# Autodesk Inventor assembly: MeasurementChamber V4 - SimulationAssembly
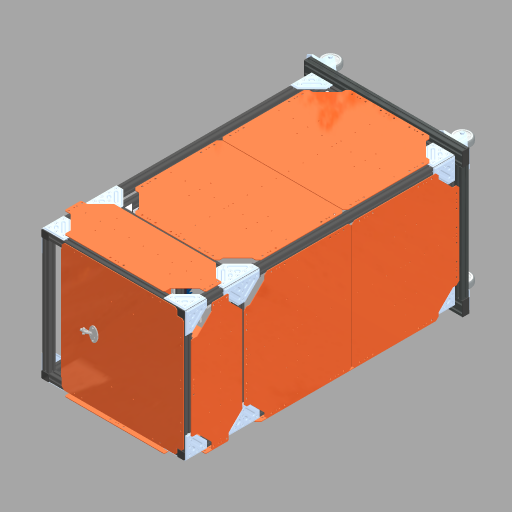
[picture p0: Inventor's stored thumbnail of the model, 512x512]
Saved by Autodesk Inventor 2023 (Build 270158000, 158)
## iProperties
Created: 2024-02-07
Part Number: MeasurementChamber V4 - SimulationAssembly
Document SubType Name: Assembly
Designer: Nils Bade
Mass: 78312.5 g
Surface Area: 384225 cm^2
Volume: 71597.2 cm^3
Density: 1.09379 g/cm^3
Author: Nils Bade
## Documents named in this file (39)
- C:\Users\Nils Bade\Documents\Projektarbeit_Bade\GIT\Masterarbeit-Inventor\RatRig_Bade\Simulation-3D-Models\MeasurementChamber V4 - SimulationAssembly.iam
- C:\Users\Nils Bade\Documents\Projektarbeit_Bade\GIT\Masterarbeit-Inventor\ITEM\ITEM Frame Assembly - Bade v1.iam
- ITEM Frame Assembly - Bade v1.iam
- C:\Users\Nils Bade\Documents\Projektarbeit_Bade\GIT\Masterarbeit-Inventor\RatRig_Bade\Z-Axis Transmission Assembly Back.iam
- C:\Users\Nils Bade\Documents\Projektarbeit_Bade\GIT\Masterarbeit-Inventor\RatRig_Bade\Z-Axis Transmission Assembly Front.iam
- C:\Users\Nils Bade\Documents\Projektarbeit_Bade\GIT\Masterarbeit-Inventor\RatRig_modified\Lead Screw - TR8x8-2p 1057mm Simple.ipt
- C:\Users\Nils Bade\Documents\Projektarbeit_Bade\GIT\Masterarbeit-Inventor\RatRig_modified\Leadscrew Constraint Front for 4040 - Assembly.iam
- C:\Users\Nils Bade\Documents\Projektarbeit_Bade\GIT\Masterarbeit-Inventor\RatRig_modified\Leadscrew Constraint Rear for 4040 - Assembly.iam
- C:\Users\Nils Bade\Documents\Projektarbeit_Bade\GIT\Masterarbeit-Inventor\RatRig_Bade\Bed Arm Back for 4040 - Assembly.iam
- C:\Users\Nils Bade\Documents\Projektarbeit_Bade\GIT\Masterarbeit-Inventor\RatRig_Bade\Bed Arm Left for 4040 - Assembly.iam
- C:\Users\Nils Bade\Documents\Projektarbeit_Bade\GIT\Masterarbeit-Inventor\RatRig_Bade\Bed Arm Right for 4040 - Assembly.iam
- C:\Users\Nils Bade\Documents\Projektarbeit_Bade\GIT\Masterarbeit-Inventor\RatRig_Bade\RatRig-Bade-BedAssembly.iam
- C:\Users\Nils Bade\Documents\Projektarbeit_Bade\GIT\Masterarbeit-Inventor\RatRig_Bade\CoreXY Idler 4040 Assembly Left V2.iam
- C:\Users\Nils Bade\Documents\Projektarbeit_Bade\GIT\Masterarbeit-Inventor\RatRig_Bade\CoreXY Idler 4040 Assembly Right V2.iam
- C:\Users\Nils Bade\Documents\Projektarbeit_Bade\GIT\Masterarbeit-Inventor\RatRig_Bade\CoreXY Motor Assembly Left for 4040 - V3.iam
- C:\Users\Nils Bade\Documents\Projektarbeit_Bade\GIT\Masterarbeit-Inventor\RatRig_Bade\CoreXY Motor Assembly Right for 4040 - V3.iam
- C:\Users\Nils Bade\Documents\Projektarbeit_Bade\GIT\Masterarbeit-Inventor\RatRig_Bade\CoreXY Belts - modified Bade.ipt
- C:\Users\Nils Bade\Documents\Projektarbeit_Bade\GIT\Masterarbeit-Inventor\RatRig_Bade\X-Gantry Assembly for 4040 V3.iam
- C:\Users\Nils Bade\Documents\Projektarbeit_Bade\GIT\Masterarbeit-Inventor\Enclosure\enc - FrontPanel Oben V2 - Assembly.iam
- C:\Users\Nils Bade\Documents\Projektarbeit_Bade\GIT\Masterarbeit-Inventor\Enclosure\enc - SidePanel Oben V2 - Assembly.iam
- C:\Users\Nils Bade\Documents\Projektarbeit_Bade\GIT\Masterarbeit-Inventor\Enclosure\enc-FrontPanel Unten - Assembly no Absorber.iam
- C:\Users\Nils Bade\Documents\Projektarbeit_Bade\GIT\Masterarbeit-Inventor\Enclosure\enc-SidePanel Unten - Assembly no Absorber.iam
- C:\Users\Nils Bade\Documents\Projektarbeit_Bade\GIT\Masterarbeit-Inventor\Enclosure\enc-BackPanel Unten - Assembly.iam
- C:\Users\Nils Bade\Documents\Projektarbeit_Bade\GIT\Masterarbeit-Inventor\Enclosure\enc-BackPanel Unten HF-Durchlass - Assembly.iam
- C:\Users\Nils Bade\Documents\Projektarbeit_Bade\GIT\Masterarbeit-Inventor\RatRig_Bade\HF-Kabelführung Measurement Chamber\HF-Kabelführung-Back-Assembly.iam
- C:\Users\Nils Bade\Documents\Projektarbeit_Bade\GIT\Masterarbeit-Inventor\Enclosure\enc-BackPanel Top V2 - Assembly.iam
- C:\Users\Nils Bade\Documents\Projektarbeit_Bade\GIT\Masterarbeit-Inventor\Enclosure\enc-TopPanel V2 - Assembly no Absorber.iam
- C:\Users\Nils Bade\Documents\Projektarbeit_Bade\GIT\Masterarbeit-Inventor\ITEM\item_kabelfuhrungsprofil-8-40_L-200mm_65445.ipt
- C:\Users\Nils Bade\Documents\Projektarbeit_Bade\GIT\Masterarbeit-Inventor\ITEM\item_kabelfuhrungsprofil-8-40_L-500mm_65445.ipt
- C:\Users\Nils Bade\Documents\Projektarbeit_Bade\GIT\Masterarbeit-Inventor\RatRig_Bade\Profile Endstop Assembly - XDirLimit.iam
- C:\Users\Nils Bade\Documents\Projektarbeit_Bade\GIT\Masterarbeit-Inventor\ITEM\item_Universal-Halter 8_0049452.ipt
- C:\Users\Nils Bade\Documents\Projektarbeit_Bade\GIT\Masterarbeit-Inventor\Enclosure\enc-ElectronicsPanel V1 - Assembly.iam
- C:\Users\Nils Bade\Documents\Projektarbeit_Bade\GIT\Masterarbeit-Inventor\RatRig_modified\ProbeHead\BLTouch-WiringSocket - Assembly.iam
- C:\Users\Nils Bade\Documents\Projektarbeit_Bade\GIT\Masterarbeit-Inventor\RatRig_Bade\HF-Kabelführung Measurement Chamber\HF-Kabelführung-V3-XGantry.iam
- C:\Users\Nils Bade\Documents\Projektarbeit_Bade\GIT\Masterarbeit-Inventor\RatRig_modified\ProbeHead\LevelingHead V1 - Assembly.iam
- C:\Users\Nils Bade\Documents\Projektarbeit_Bade\GIT\Masterarbeit-Inventor\RatRig_Bade\MeasurementChamber RollBase V1.iam
- C:\Users\Nils Bade\Documents\Projektarbeit_Bade\GIT\Masterarbeit-Inventor\RatRig_modified\Chamber_BauteilHaken.iam
- C:\Users\Nils Bade\Documents\Projektarbeit_Bade\GIT\Masterarbeit-Inventor\AUT-Mountings\AUT_60GHz_Horn_Mounted.iam
- C:\Users\Nils Bade\Documents\Projektarbeit_Bade\GIT\Masterarbeit-Inventor\RatRig_modified\ProbeHead\ProbeHead V5 - Assembly.iam
## Components (56 placed, 37 different names)
1. ITEM Frame Assembly - Bade v1:1 [sub-assembly] — Passend:1, Passend:2, Passend:3, Passend:4, Passend:5, Passend:6, Passend:7, Passend:8, Passend:9, Passend:10, Passend:11, Passend:12, Passend:16, Passend:17, Passend:18, Passend:19, Passend:20, Passend:21, Passend:22, Fluchtend:3, Fluchtend:4, Passend:23, Passend:24, Passend:26, Passend:27, Passend:28, Passend:30, Passend:31, Passend:32, Passend:33, Passend:34, Passend:35, Passend:36, Passend:37, Passend:38, Passend:39, Passend:40, Passend:41, Fluchtend:7, Fluchtend:8, Passend:46, Fluchtend:9, Fluchtend:10, Fluchtend:11, Passend:47, Fluchtend:12, Fluchtend:13, Passend:48, Passend:49, Passend:50, Passend:51, Passend:52, Passend:53, Fluchtend:14, Fluchtend:15, Fluchtend:16, Passend:54, Passend:55, Passend:56, Passend:57, Passend:58, Passend:59, Passend:60, Fluchtend:17, Passend:61, Fluchtend:18, Fluchtend:19, Passend:62, Passend:63, Passend:64, Passend:65, Passend:66, Passend:67, Fluchtend:20, Fluchtend:21, Fluchtend:22, Passend:68, Fluchtend:23, Fluchtend:24, Passend:69, Passend:70, Passend:71, Fluchtend:25, Fluchtend:26, Passend:72, Passend:73, Passend:74, Passend:75, Passend:76, Fluchtend:27, Passend:77, Passend:78, Passend:80, Passend:81, Passend:82, Passend:83, Passend:84, Passend:85, Fluchtend:28, Fluchtend:29, Passend:86, Passend:87, Passend:95, Passend:96, Fluchtend:32, Passend:98, Passend:100, Passend:101, Passend:103, Passend:104, Passend:105, Fluchtend:33, Passend:106, Fluchtend:110, Passend:113, Passend:114, Passend:115, Passend:116, Passend:117, Passend:118, Passend:119, Passend:120, Passend:121, Passend:122, Fluchtend:111, Passend:123, Passend:124, Fluchtend:112, Passend:125, Passend:126, Fluchtend:113, Passend:138, Passend:130, Winkel:1, Fluchtend:115, Fluchtend:116, Fluchtend:117, Passend:136, Passend:137, Fluchtend:118, Passend:139, Passend:140, Passend:141, Fluchtend:120, Passend:143, Passend:144, Fluchtend:121
2. RatRig-Bade-BedAssembly:1 [sub-assembly] — Passend:27, Passend:28, Passend:29, Passend:145, Passend:146, FLUCHTEND-PLATE-HEAD
3. MeasurementChamber RollBase V1:1 [sub-assembly] — Passend:139, Passend:140, Passend:141
4. AUT_60GHz_Horn_Mounted:1 [sub-assembly] — Passend:145, Winkel:2, Passend:146
5. Z-Axis Transmission Assembly Back:1 [sub-assembly] — Passend:1, Passend:2, Passend:3, Passend:15, Passend:97
6. Z-Axis Transmission Assembly Front:1 [sub-assembly] — Passend:4, Passend:5, Passend:6, Passend:14, Passend:102
7. Z-Axis Transmission Assembly Front:2 [sub-assembly] — Passend:7, Passend:8, Passend:9, Passend:13, Passend:99
8. LeadScrew - TR8x8-2p 1057mm Simple:1 — Passend:10, Passend:15, Passend:25
9. LeadScrew - TR8x8-2p 1057mm Simple:2 — Passend:11, Passend:14
10. LeadScrew - TR8x8-2p 1057mm Simple:3 — Passend:12, Passend:13
11. Leadscrew Constraint Front for 4040 - Assembly:1 [sub-assembly] — Passend:16, Passend:19, Fluchtend:1, Passend:22
12. Leadscrew Constraint Front for 4040 - Assembly:2 [sub-assembly] — Passend:17, Passend:18, Fluchtend:1, Fluchtend:2
13. Leadscrew Constraint Rear for 4040 - Assembly:1 [sub-assembly] — Passend:20, Passend:21, Fluchtend:2
14. Bed Arm Back for 4040 - Assembly:1 [sub-assembly] — Fluchtend:3, Fluchtend:6, Passend:25, Passend:29
15. Bed Arm Left for 4040 - Assembly:1 [sub-assembly] — Passend:23, Fluchtend:5, Fluchtend:6, Passend:26
16. Bed Arm Right for 4040 - Assembly:1 [sub-assembly] — Fluchtend:4, Fluchtend:5, Passend:24
17. Profile Endstop Assembly - XDirLimit:1 [sub-assembly] — Fluchtend:110, Passend:113, Passend:114
18. CoreXY Idler 4040 Assembly Left V2:1 [sub-assembly] — Passend:33, Passend:34, Passend:35
19. CoreXY Idler 4040 Assembly Right V2:1 [sub-assembly] — Passend:30, Passend:31, Passend:32, Passend:44, Passend:45
20. CoreXY Motor Assembly Left for 4040 - V3:1 [sub-assembly] — Passend:36, Passend:37, Passend:38, Passend:42
21. CoreXY Motor Assembly Right for 4040 - V3:1 [sub-assembly] — Passend:39, Passend:40, Passend:41, Passend:43
22. CoreXY Belts - modified Bade:1 — Passend:42, Passend:43, Passend:44, Passend:45, Passend:142
23. X-Gantry Assembly for 4040 V3:1 [sub-assembly] — Fluchtend:7, Fluchtend:8, Passend:46, Passend:142
24. ProbeHead V3 - Assembly:2 [sub-assembly]
25. ProbeHead V5 - Assembly:1 [sub-assembly] — FLUCHTEND-PLATE-HEAD
26. enc-TopPanel V2 - Assembly no Absorber:1 [sub-assembly] — Fluchtend:29, Passend:86, Passend:87, Passend:133
27. enc-BackPanel Top V2 - Assembly:1 [sub-assembly] — Passend:83, Passend:84, Passend:85, Fluchtend:28
28. enc-FrontPanel Oben V2 - Assembly:1 [sub-assembly] — Fluchtend:9, Fluchtend:10, Fluchtend:11, Passend:47
29. enc-SidePanel Oben V2 - Assembly:1 [sub-assembly] — Fluchtend:12, Fluchtend:13, Passend:48, Passend:49
30. enc-SidePanel Oben V2 - Assembly:2 [sub-assembly] — Passend:50, Passend:51, Passend:52, Passend:53
31. enc-FrontPanel Unten - Assembly no Absorber:1 [sub-assembly] — Passend:55, Passend:56, Passend:57, Passend:58
32. enc-FrontPanel Unten - Assembly no Absorber:2 [sub-assembly] — Fluchtend:14, Fluchtend:15, Fluchtend:16, Passend:54
33. enc-SidePanel Unten - Assembly no Absorber:1 [sub-assembly] — Fluchtend:20, Fluchtend:21, Fluchtend:22, Passend:68
34. enc-SidePanel Unten - Assembly no Absorber:2 [sub-assembly] — Passend:64, Passend:65, Passend:66, Passend:67
35. enc-SidePanel Unten - Assembly no Absorber:3 [sub-assembly] — Fluchtend:18, Fluchtend:19, Passend:62, Passend:63
36. enc-SidePanel Unten - Assembly no Absorber:4 [sub-assembly] — Passend:59, Passend:60, Fluchtend:17, Passend:61
37. enc-BackPanel Unten - Assembly:1 [sub-assembly] — Fluchtend:26, Passend:72, Passend:73, Passend:76
38. enc-BackPanel Unten - Assembly:2 [sub-assembly] — Fluchtend:25, Passend:74, Passend:75
39. enc-BackPanel Unten - Assembly:3 [sub-assembly] — Fluchtend:24, Passend:69, Passend:70, Passend:71
40. enc-BackPanel Unten HF-Durchlass - Assembly:1 [sub-assembly] — Fluchtend:27, Passend:77, Passend:78
41. HF-Kabelführung-Back-Assembly:1 [sub-assembly] — Passend:79, Passend:80, Passend:81, Passend:82
42. HF-Kabelführung-V3-XGantry:1 [sub-assembly] — Winkel:1, Passend:133, Fluchtend:115, Fluchtend:116
43. BLTouch-WiringSocket - Assembly:1 [sub-assembly] — Passend:138, Passend:130, Fluchtend:118
44. enc-ElectronicsPanel V1 - Assembly:1 [sub-assembly] — Fluchtend:117, Passend:136, Passend:137
45. item_kabelfuhrungsprofil-8-40_L-200mm_65445:1 — Passend:95, Passend:96, Passend:97
46. item_kabelfuhrungsprofil-8-40_L-500mm_65445:1 — Fluchtend:32, Passend:98, Passend:99
47. item_kabelfuhrungsprofil-8-40_L-500mm_65445:2 — Passend:100, Passend:101, Passend:102
48. item_kabelfuhrungsprofil-8-40_L-500mm_65445:3 — Passend:103, Passend:105, Fluchtend:33, Passend:107
49. item_kabelfuhrungsprofil-8-40_L-500mm_65445:4 — Passend:104, Passend:106, Passend:107
50. Chamber_BauteilHaken:1 [sub-assembly] — Fluchtend:120, Passend:143
51. Chamber_BauteilHaken:2 [sub-assembly] — Passend:144, Fluchtend:121
52. item_kabelfuhrungsprofil-8-40_L-200mm_65445:2 — Passend:118, Passend:121, Passend:122
53. item_kabelfuhrungsprofil-8-40_L-200mm_65445:3 — Passend:119, Passend:120, Fluchtend:111
54. item_Universal-Halter 8_0049452:1 — Passend:115, Passend:116, Passend:117
55. item_Universal-Halter 8_0049452:3 — Passend:125, Passend:126, Fluchtend:113
56. item_Universal-Halter 8_0049452:2 — Passend:123, Passend:124, Fluchtend:112
## Relationships (178: Mate 132, Flush 44, Angle 2)
- Passend:1 [Mate]: ITEM Frame Assembly - Bade v1:1 ↔ Z-Axis Transmission Assembly Back:1
- Passend:2 [Mate]: ITEM Frame Assembly - Bade v1:1 ↔ Z-Axis Transmission Assembly Back:1
- Passend:3 [Mate]: ITEM Frame Assembly - Bade v1:1 ↔ Z-Axis Transmission Assembly Back:1
- Passend:4 [Mate]: ITEM Frame Assembly - Bade v1:1 ↔ Z-Axis Transmission Assembly Front:1
- Passend:5 [Mate]: ITEM Frame Assembly - Bade v1:1 ↔ Z-Axis Transmission Assembly Front:1
- Passend:6 [Mate]: ITEM Frame Assembly - Bade v1:1 ↔ Z-Axis Transmission Assembly Front:1
- Passend:7 [Mate]: ITEM Frame Assembly - Bade v1:1 ↔ Z-Axis Transmission Assembly Front:2
- Passend:8 [Mate]: ITEM Frame Assembly - Bade v1:1 ↔ Z-Axis Transmission Assembly Front:2
- Passend:9 [Mate]: ITEM Frame Assembly - Bade v1:1 ↔ Z-Axis Transmission Assembly Front:2
- Passend:10 [Mate]: ITEM Frame Assembly - Bade v1:1 ↔ LeadScrew - TR8x8-2p 1057mm Simple:1
- Passend:11 [Mate]: ITEM Frame Assembly - Bade v1:1 ↔ LeadScrew - TR8x8-2p 1057mm Simple:2
- Passend:12 [Mate]: ITEM Frame Assembly - Bade v1:1 ↔ LeadScrew - TR8x8-2p 1057mm Simple:3
- Passend:13 [Mate]: Z-Axis Transmission Assembly Front:2 ↔ LeadScrew - TR8x8-2p 1057mm Simple:3
- Passend:14 [Mate]: Z-Axis Transmission Assembly Front:1 ↔ LeadScrew - TR8x8-2p 1057mm Simple:2
- Passend:15 [Mate]: Z-Axis Transmission Assembly Back:1 ↔ LeadScrew - TR8x8-2p 1057mm Simple:1
- Passend:16 [Mate]: ITEM Frame Assembly - Bade v1:1 ↔ Leadscrew Constraint Front for 4040 - Assembly:1
- Passend:17 [Mate]: ITEM Frame Assembly - Bade v1:1 ↔ Leadscrew Constraint Front for 4040 - Assembly:2
- Passend:18 [Mate]: ITEM Frame Assembly - Bade v1:1 ↔ Leadscrew Constraint Front for 4040 - Assembly:2
- Passend:19 [Mate]: ITEM Frame Assembly - Bade v1:1 ↔ Leadscrew Constraint Front for 4040 - Assembly:1
- Fluchtend:1 [Flush]: Leadscrew Constraint Front for 4040 - Assembly:1 ↔ Leadscrew Constraint Front for 4040 - Assembly:2
- Passend:20 [Mate]: ITEM Frame Assembly - Bade v1:1 ↔ Leadscrew Constraint Rear for 4040 - Assembly:1
- Passend:21 [Mate]: ITEM Frame Assembly - Bade v1:1 ↔ Leadscrew Constraint Rear for 4040 - Assembly:1
- Fluchtend:2 [Flush]: Leadscrew Constraint Front for 4040 - Assembly:2 ↔ Leadscrew Constraint Rear for 4040 - Assembly:1
- Passend:22 [Mate] (5 mm): ITEM Frame Assembly - Bade v1:1 ↔ Leadscrew Constraint Front for 4040 - Assembly:1
- Fluchtend:3 [Flush]: ITEM Frame Assembly - Bade v1:1 ↔ Bed Arm Back for 4040 - Assembly:1
- Fluchtend:4 [Flush]: ITEM Frame Assembly - Bade v1:1 ↔ Bed Arm Right for 4040 - Assembly:1
- Passend:23 [Mate]: ITEM Frame Assembly - Bade v1:1 ↔ Bed Arm Left for 4040 - Assembly:1
- Fluchtend:5 [Flush]: Bed Arm Left for 4040 - Assembly:1 ↔ Bed Arm Right for 4040 - Assembly:1
- Fluchtend:6 [Flush]: Bed Arm Back for 4040 - Assembly:1 ↔ Bed Arm Left for 4040 - Assembly:1
- Passend:24 [Mate]: ITEM Frame Assembly - Bade v1:1 ↔ Bed Arm Right for 4040 - Assembly:1
- Passend:25 [Mate]: LeadScrew - TR8x8-2p 1057mm Simple:1 ↔ Bed Arm Back for 4040 - Assembly:1
- Passend:26 [Mate]: ITEM Frame Assembly - Bade v1:1 ↔ Bed Arm Left for 4040 - Assembly:1
- Passend:27 [Mate]: ITEM Frame Assembly - Bade v1:1 ↔ RatRig-Bade-BedAssembly:1
- Passend:28 [Mate] (12.5 mm): ITEM Frame Assembly - Bade v1:1 ↔ RatRig-Bade-BedAssembly:1
- Passend:29 [Mate] (11.5 mm): RatRig-Bade-BedAssembly:1 ↔ Bed Arm Back for 4040 - Assembly:1
- Passend:30 [Mate]: ITEM Frame Assembly - Bade v1:1 ↔ CoreXY Idler 4040 Assembly Right V2:1
- Passend:31 [Mate]: ITEM Frame Assembly - Bade v1:1 ↔ CoreXY Idler 4040 Assembly Right V2:1
- Passend:32 [Mate]: ITEM Frame Assembly - Bade v1:1 ↔ CoreXY Idler 4040 Assembly Right V2:1
- Passend:33 [Mate]: ITEM Frame Assembly - Bade v1:1 ↔ CoreXY Idler 4040 Assembly Left V2:1
- Passend:34 [Mate]: ITEM Frame Assembly - Bade v1:1 ↔ CoreXY Idler 4040 Assembly Left V2:1
- Passend:35 [Mate]: ITEM Frame Assembly - Bade v1:1 ↔ CoreXY Idler 4040 Assembly Left V2:1
- Passend:36 [Mate]: ITEM Frame Assembly - Bade v1:1 ↔ CoreXY Motor Assembly Left for 4040 - V3:1
- Passend:37 [Mate]: ITEM Frame Assembly - Bade v1:1 ↔ CoreXY Motor Assembly Left for 4040 - V3:1
- Passend:38 [Mate]: ITEM Frame Assembly - Bade v1:1 ↔ CoreXY Motor Assembly Left for 4040 - V3:1
- Passend:39 [Mate]: ITEM Frame Assembly - Bade v1:1 ↔ CoreXY Motor Assembly Right for 4040 - V3:1
- Passend:40 [Mate]: ITEM Frame Assembly - Bade v1:1 ↔ CoreXY Motor Assembly Right for 4040 - V3:1
- Passend:41 [Mate]: ITEM Frame Assembly - Bade v1:1 ↔ CoreXY Motor Assembly Right for 4040 - V3:1
- Passend:42 [Mate]: CoreXY Motor Assembly Left for 4040 - V3:1 ↔ CoreXY Belts - modified Bade:1
- Passend:43 [Mate]: CoreXY Motor Assembly Right for 4040 - V3:1 ↔ CoreXY Belts - modified Bade:1
- Passend:44 [Mate]: CoreXY Idler 4040 Assembly Right V2:1 ↔ CoreXY Belts - modified Bade:1
- Passend:45 [Mate] (0.5 mm): CoreXY Idler 4040 Assembly Right V2:1 ↔ CoreXY Belts - modified Bade:1
- Fluchtend:7 [Flush]: ITEM Frame Assembly - Bade v1:1 ↔ X-Gantry Assembly for 4040 V3:1
- Fluchtend:8 [Flush]: ITEM Frame Assembly - Bade v1:1 ↔ X-Gantry Assembly for 4040 V3:1
- Passend:46 [Mate]: ITEM Frame Assembly - Bade v1:1 ↔ X-Gantry Assembly for 4040 V3:1
- Fluchtend:9 [Flush]: ITEM Frame Assembly - Bade v1:1 ↔ enc-FrontPanel Oben V2 - Assembly:1
- Fluchtend:10 [Flush]: ITEM Frame Assembly - Bade v1:1 ↔ enc-FrontPanel Oben V2 - Assembly:1
- Fluchtend:11 [Flush]: ITEM Frame Assembly - Bade v1:1 ↔ enc-FrontPanel Oben V2 - Assembly:1
- Passend:47 [Mate]: ITEM Frame Assembly - Bade v1:1 ↔ enc-FrontPanel Oben V2 - Assembly:1
- Fluchtend:12 [Flush]: ITEM Frame Assembly - Bade v1:1 ↔ enc-SidePanel Oben V2 - Assembly:1
- Fluchtend:13 [Flush]: ITEM Frame Assembly - Bade v1:1 ↔ enc-SidePanel Oben V2 - Assembly:1
- Passend:48 [Mate]: ITEM Frame Assembly - Bade v1:1 ↔ enc-SidePanel Oben V2 - Assembly:1
- Passend:49 [Mate]: ITEM Frame Assembly - Bade v1:1 ↔ enc-SidePanel Oben V2 - Assembly:1
- Passend:50 [Mate]: ITEM Frame Assembly - Bade v1:1 ↔ enc-SidePanel Oben V2 - Assembly:2
- Passend:51 [Mate]: ITEM Frame Assembly - Bade v1:1 ↔ enc-SidePanel Oben V2 - Assembly:2
- Passend:52 [Mate]: ITEM Frame Assembly - Bade v1:1 ↔ enc-SidePanel Oben V2 - Assembly:2
- Passend:53 [Mate]: ITEM Frame Assembly - Bade v1:1 ↔ enc-SidePanel Oben V2 - Assembly:2
- Fluchtend:14 [Flush]: ITEM Frame Assembly - Bade v1:1 ↔ enc-FrontPanel Unten - Assembly no Absorber:2
- Fluchtend:15 [Flush]: ITEM Frame Assembly - Bade v1:1 ↔ enc-FrontPanel Unten - Assembly no Absorber:2
- Fluchtend:16 [Flush]: ITEM Frame Assembly - Bade v1:1 ↔ enc-FrontPanel Unten - Assembly no Absorber:2
- Passend:54 [Mate]: ITEM Frame Assembly - Bade v1:1 ↔ enc-FrontPanel Unten - Assembly no Absorber:2
- Passend:55 [Mate]: ITEM Frame Assembly - Bade v1:1 ↔ enc-FrontPanel Unten - Assembly no Absorber:1
- Passend:56 [Mate]: ITEM Frame Assembly - Bade v1:1 ↔ enc-FrontPanel Unten - Assembly no Absorber:1
- Passend:57 [Mate]: ITEM Frame Assembly - Bade v1:1 ↔ enc-FrontPanel Unten - Assembly no Absorber:1
- Passend:58 [Mate]: ITEM Frame Assembly - Bade v1:1 ↔ enc-FrontPanel Unten - Assembly no Absorber:1
- Passend:59 [Mate]: ITEM Frame Assembly - Bade v1:1 ↔ enc-SidePanel Unten - Assembly no Absorber:4
- Passend:60 [Mate]: ITEM Frame Assembly - Bade v1:1 ↔ enc-SidePanel Unten - Assembly no Absorber:4
- Fluchtend:17 [Flush]: ITEM Frame Assembly - Bade v1:1 ↔ enc-SidePanel Unten - Assembly no Absorber:4
- Passend:61 [Mate]: ITEM Frame Assembly - Bade v1:1 ↔ enc-SidePanel Unten - Assembly no Absorber:4
- Fluchtend:18 [Flush]: ITEM Frame Assembly - Bade v1:1 ↔ enc-SidePanel Unten - Assembly no Absorber:3
- Fluchtend:19 [Flush]: ITEM Frame Assembly - Bade v1:1 ↔ enc-SidePanel Unten - Assembly no Absorber:3
- Passend:62 [Mate]: ITEM Frame Assembly - Bade v1:1 ↔ enc-SidePanel Unten - Assembly no Absorber:3
- Passend:63 [Mate]: ITEM Frame Assembly - Bade v1:1 ↔ enc-SidePanel Unten - Assembly no Absorber:3
- Passend:64 [Mate]: ITEM Frame Assembly - Bade v1:1 ↔ enc-SidePanel Unten - Assembly no Absorber:2
- Passend:65 [Mate]: ITEM Frame Assembly - Bade v1:1 ↔ enc-SidePanel Unten - Assembly no Absorber:2
- Passend:66 [Mate]: ITEM Frame Assembly - Bade v1:1 ↔ enc-SidePanel Unten - Assembly no Absorber:2
- Passend:67 [Mate]: ITEM Frame Assembly - Bade v1:1 ↔ enc-SidePanel Unten - Assembly no Absorber:2
- Fluchtend:20 [Flush]: ITEM Frame Assembly - Bade v1:1 ↔ enc-SidePanel Unten - Assembly no Absorber:1
- Fluchtend:21 [Flush]: ITEM Frame Assembly - Bade v1:1 ↔ enc-SidePanel Unten - Assembly no Absorber:1
- Fluchtend:22 [Flush]: ITEM Frame Assembly - Bade v1:1 ↔ enc-SidePanel Unten - Assembly no Absorber:1
- Passend:68 [Mate]: ITEM Frame Assembly - Bade v1:1 ↔ enc-SidePanel Unten - Assembly no Absorber:1
- Fluchtend:23 [Flush] (800 mm): ITEM Frame Assembly - Bade v1:1
- Fluchtend:24 [Flush]: ITEM Frame Assembly - Bade v1:1 ↔ enc-BackPanel Unten - Assembly:3
- Passend:69 [Mate]: ITEM Frame Assembly - Bade v1:1 ↔ enc-BackPanel Unten - Assembly:3
- Passend:70 [Mate]: ITEM Frame Assembly - Bade v1:1 ↔ enc-BackPanel Unten - Assembly:3
- Passend:71 [Mate]: ITEM Frame Assembly - Bade v1:1 ↔ enc-BackPanel Unten - Assembly:3
- Fluchtend:25 [Flush]: ITEM Frame Assembly - Bade v1:1 ↔ enc-BackPanel Unten - Assembly:2
- Fluchtend:26 [Flush]: ITEM Frame Assembly - Bade v1:1 ↔ enc-BackPanel Unten - Assembly:1
- Passend:72 [Mate]: ITEM Frame Assembly - Bade v1:1 ↔ enc-BackPanel Unten - Assembly:1
- Passend:73 [Mate]: ITEM Frame Assembly - Bade v1:1 ↔ enc-BackPanel Unten - Assembly:1
- Passend:74 [Mate]: ITEM Frame Assembly - Bade v1:1 ↔ enc-BackPanel Unten - Assembly:2
- Passend:75 [Mate]: ITEM Frame Assembly - Bade v1:1 ↔ enc-BackPanel Unten - Assembly:2
- Passend:76 [Mate]: ITEM Frame Assembly - Bade v1:1 ↔ enc-BackPanel Unten - Assembly:1
- Fluchtend:27 [Flush]: ITEM Frame Assembly - Bade v1:1 ↔ enc-BackPanel Unten HF-Durchlass - Assembly:1
- Passend:77 [Mate]: ITEM Frame Assembly - Bade v1:1 ↔ enc-BackPanel Unten HF-Durchlass - Assembly:1
- Passend:78 [Mate]: ITEM Frame Assembly - Bade v1:1 ↔ enc-BackPanel Unten HF-Durchlass - Assembly:1
- Passend:79 [Mate]: HF-Kabelführung-Back-Assembly:1
- Passend:80 [Mate]: ITEM Frame Assembly - Bade v1:1 ↔ HF-Kabelführung-Back-Assembly:1
- Passend:81 [Mate]: ITEM Frame Assembly - Bade v1:1 ↔ HF-Kabelführung-Back-Assembly:1
- Passend:82 [Mate]: ITEM Frame Assembly - Bade v1:1 ↔ HF-Kabelführung-Back-Assembly:1
- Passend:83 [Mate]: ITEM Frame Assembly - Bade v1:1 ↔ enc-BackPanel Top V2 - Assembly:1
- Passend:84 [Mate]: ITEM Frame Assembly - Bade v1:1 ↔ enc-BackPanel Top V2 - Assembly:1
- Passend:85 [Mate]: ITEM Frame Assembly - Bade v1:1 ↔ enc-BackPanel Top V2 - Assembly:1
- Fluchtend:28 [Flush]: ITEM Frame Assembly - Bade v1:1 ↔ enc-BackPanel Top V2 - Assembly:1
- Fluchtend:29 [Flush]: ITEM Frame Assembly - Bade v1:1 ↔ enc-TopPanel V2 - Assembly no Absorber:1
- Passend:86 [Mate]: ITEM Frame Assembly - Bade v1:1 ↔ enc-TopPanel V2 - Assembly no Absorber:1
- Passend:87 [Mate]: ITEM Frame Assembly - Bade v1:1 ↔ enc-TopPanel V2 - Assembly no Absorber:1
- Passend:95 [Mate]: ITEM Frame Assembly - Bade v1:1 ↔ item_kabelfuhrungsprofil-8-40_L-200mm_65445:1
- Passend:96 [Mate]: ITEM Frame Assembly - Bade v1:1 ↔ item_kabelfuhrungsprofil-8-40_L-200mm_65445:1
- Passend:97 [Mate] (40 mm): Z-Axis Transmission Assembly Back:1 ↔ item_kabelfuhrungsprofil-8-40_L-200mm_65445:1
- Fluchtend:32 [Flush]: ITEM Frame Assembly - Bade v1:1 ↔ item_kabelfuhrungsprofil-8-40_L-500mm_65445:1
- Passend:98 [Mate]: ITEM Frame Assembly - Bade v1:1 ↔ item_kabelfuhrungsprofil-8-40_L-500mm_65445:1
- Passend:99 [Mate] (25 mm): Z-Axis Transmission Assembly Front:2 ↔ item_kabelfuhrungsprofil-8-40_L-500mm_65445:1
- Passend:100 [Mate]: ITEM Frame Assembly - Bade v1:1 ↔ item_kabelfuhrungsprofil-8-40_L-500mm_65445:2
- Passend:101 [Mate]: ITEM Frame Assembly - Bade v1:1 ↔ item_kabelfuhrungsprofil-8-40_L-500mm_65445:2
- Passend:102 [Mate] (30 mm): Z-Axis Transmission Assembly Front:1 ↔ item_kabelfuhrungsprofil-8-40_L-500mm_65445:2
- Passend:103 [Mate]: ITEM Frame Assembly - Bade v1:1 ↔ item_kabelfuhrungsprofil-8-40_L-500mm_65445:3
- Passend:104 [Mate]: ITEM Frame Assembly - Bade v1:1 ↔ item_kabelfuhrungsprofil-8-40_L-500mm_65445:4
- Passend:105 [Mate]: ITEM Frame Assembly - Bade v1:1 ↔ item_kabelfuhrungsprofil-8-40_L-500mm_65445:3
- Fluchtend:33 [Flush]: ITEM Frame Assembly - Bade v1:1 ↔ item_kabelfuhrungsprofil-8-40_L-500mm_65445:3
- Passend:106 [Mate]: ITEM Frame Assembly - Bade v1:1 ↔ item_kabelfuhrungsprofil-8-40_L-500mm_65445:4
- Passend:107 [Mate]: item_kabelfuhrungsprofil-8-40_L-500mm_65445:3 ↔ item_kabelfuhrungsprofil-8-40_L-500mm_65445:4
- [Mate]: X-Gantry Assembly for 4040 V3:1 ↔ ProbeHead V3 - Assembly:2
- [Mate]: X-Gantry Assembly for 4040 V3:1 ↔ ProbeHead V3 - Assembly:2
- Fluchtend:110 [Flush]: ITEM Frame Assembly - Bade v1:1 ↔ Profile Endstop Assembly - XDirLimit:1
- Passend:113 [Mate]: ITEM Frame Assembly - Bade v1:1 ↔ Profile Endstop Assembly - XDirLimit:1
- Passend:114 [Mate] (5 mm): ITEM Frame Assembly - Bade v1:1 ↔ Profile Endstop Assembly - XDirLimit:1
- Passend:115 [Mate]: ITEM Frame Assembly - Bade v1:1 ↔ item_Universal-Halter 8_0049452:1
- Passend:116 [Mate]: ITEM Frame Assembly - Bade v1:1 ↔ item_Universal-Halter 8_0049452:1
- Passend:117 [Mate] (20 mm): ITEM Frame Assembly - Bade v1:1 ↔ item_Universal-Halter 8_0049452:1
- Passend:118 [Mate]: ITEM Frame Assembly - Bade v1:1 ↔ item_kabelfuhrungsprofil-8-40_L-200mm_65445:2
- Passend:119 [Mate]: ITEM Frame Assembly - Bade v1:1 ↔ item_kabelfuhrungsprofil-8-40_L-200mm_65445:3
- Passend:120 [Mate]: ITEM Frame Assembly - Bade v1:1 ↔ item_kabelfuhrungsprofil-8-40_L-200mm_65445:3
- Passend:121 [Mate]: ITEM Frame Assembly - Bade v1:1 ↔ item_kabelfuhrungsprofil-8-40_L-200mm_65445:2
- Passend:122 [Mate] (30 mm): ITEM Frame Assembly - Bade v1:1 ↔ item_kabelfuhrungsprofil-8-40_L-200mm_65445:2
- Fluchtend:111 [Flush] (30 mm): ITEM Frame Assembly - Bade v1:1 ↔ item_kabelfuhrungsprofil-8-40_L-200mm_65445:3
- Passend:123 [Mate]: ITEM Frame Assembly - Bade v1:1 ↔ item_Universal-Halter 8_0049452:2
- Passend:124 [Mate]: ITEM Frame Assembly - Bade v1:1 ↔ item_Universal-Halter 8_0049452:2
- Fluchtend:112 [Flush] (30 mm): ITEM Frame Assembly - Bade v1:1 ↔ item_Universal-Halter 8_0049452:2
- Passend:125 [Mate]: ITEM Frame Assembly - Bade v1:1 ↔ item_Universal-Halter 8_0049452:3
- Passend:126 [Mate]: ITEM Frame Assembly - Bade v1:1 ↔ item_Universal-Halter 8_0049452:3
- Fluchtend:113 [Flush] (-3 mm): ITEM Frame Assembly - Bade v1:1 ↔ item_Universal-Halter 8_0049452:3
- Passend:138 [Mate]: ITEM Frame Assembly - Bade v1:1 ↔ BLTouch-WiringSocket - Assembly:1
- Passend:130 [Mate]: ITEM Frame Assembly - Bade v1:1 ↔ BLTouch-WiringSocket - Assembly:1
- Winkel:1 [Angle] (0 deg): ITEM Frame Assembly - Bade v1:1 ↔ HF-Kabelführung-V3-XGantry:1
- Passend:133 [Mate]: enc-TopPanel V2 - Assembly no Absorber:1 ↔ HF-Kabelführung-V3-XGantry:1
- Fluchtend:115 [Flush]: ITEM Frame Assembly - Bade v1:1 ↔ HF-Kabelführung-V3-XGantry:1
- Fluchtend:116 [Flush]: ITEM Frame Assembly - Bade v1:1 ↔ HF-Kabelführung-V3-XGantry:1
- Fluchtend:117 [Flush]: ITEM Frame Assembly - Bade v1:1 ↔ enc-ElectronicsPanel V1 - Assembly:1
- Passend:136 [Mate]: ITEM Frame Assembly - Bade v1:1 ↔ enc-ElectronicsPanel V1 - Assembly:1
- Passend:137 [Mate]: ITEM Frame Assembly - Bade v1:1 ↔ enc-ElectronicsPanel V1 - Assembly:1
- Fluchtend:118 [Flush]: ITEM Frame Assembly - Bade v1:1 ↔ BLTouch-WiringSocket - Assembly:1
- Fluchtend:119 [Flush] (-170 mm)
- Passend:139 [Mate]: ITEM Frame Assembly - Bade v1:1 ↔ MeasurementChamber RollBase V1:1
- Passend:140 [Mate]: ITEM Frame Assembly - Bade v1:1 ↔ MeasurementChamber RollBase V1:1
- Passend:141 [Mate]: ITEM Frame Assembly - Bade v1:1 ↔ MeasurementChamber RollBase V1:1
- Passend:142 [Mate]: CoreXY Belts - modified Bade:1 ↔ X-Gantry Assembly for 4040 V3:1
- Fluchtend:120 [Flush]: ITEM Frame Assembly - Bade v1:1 ↔ Chamber_BauteilHaken:1
- Passend:143 [Mate]: ITEM Frame Assembly - Bade v1:1 ↔ Chamber_BauteilHaken:1
- Passend:144 [Mate]: ITEM Frame Assembly - Bade v1:1 ↔ Chamber_BauteilHaken:2
- Fluchtend:121 [Flush]: ITEM Frame Assembly - Bade v1:1 ↔ Chamber_BauteilHaken:2
- Passend:145 [Mate]: RatRig-Bade-BedAssembly:1 ↔ AUT_60GHz_Horn_Mounted:1
- Winkel:2 [Angle] (90 deg): AUT_60GHz_Horn_Mounted:1
- Passend:146 [Mate]: RatRig-Bade-BedAssembly:1 ↔ AUT_60GHz_Horn_Mounted:1
- [Mate]: X-Gantry Assembly for 4040 V3:1 ↔ ProbeHead V5 - Assembly:1
- [Mate]: X-Gantry Assembly for 4040 V3:1 ↔ ProbeHead V5 - Assembly:1
- FLUCHTEND-PLATE-HEAD [Flush] (200 mm): RatRig-Bade-BedAssembly:1 ↔ ProbeHead V5 - Assembly:1
- [Flush] (-360 mm): ProbeHead V5 - Assembly:1
- [Mate]: RatRig-Bade-BedAssembly:1 ↔ ProbeHead V5 - Assembly:1
